# Autodesk Inventor assembly: スプリング
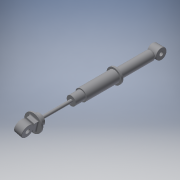
[picture p0: Inventor's stored thumbnail of the model, 180x180]
Saved by Autodesk Inventor 2018 (Build 220112000, 112)
## iProperties
Created: 2017-09-09
Part Number: スプリング
Material: 一般
Document SubType Name: Assembly
Designer: Kenta
Author: Kenta
## Documents named in this file (3)
- C:\Users\mura5\Documents\RBBR\cart\スプリング.iam
- C:\Users\mura5\Documents\RBBR\cart\スプリングその１.ipt
- C:\Users\mura5\Documents\RBBR\cart\スプリングその２.ipt
## Components (2 placed, 2 different names)
1. スプリングその１:1 — メイト:1, メイト:2
2. スプリングその２:1 — メイト:1, メイト:2
## Relationships (2: Mate 2)
- メイト:1 [Mate]: スプリングその１:1 ↔ スプリングその２:1
- メイト:2 [Mate]: スプリングその１:1 ↔ スプリングその２:1
